# Autodesk Inventor assembly: RspCameraMia_cam_alone
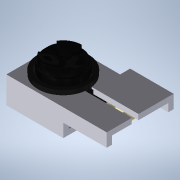
[picture p0: Inventor's stored thumbnail of the model, 180x180]
Saved by Autodesk Inventor 2020.2 (Build 242310000, 310)
## iProperties
Created: 2018-02-03
Part Number: RspCameraMia_cam_alone
Material: Genérico
Document SubType Name: Assembly
Designer: RafaX
Author: RafaX
## Documents named in this file (6)
- D:\gdrive\documents\flexipod\modelingv3\raspberry-pi-camera-module-v2-1\RspCameraMia_cam_alone.iam
- D:\gdrive\documents\flexipod\modelingv3\raspberry-pi-camera-module-v2-1\OVA5647_Housing.ipt
- D:\gdrive\documents\flexipod\modelingv3\raspberry-pi-camera-module-v2-1\OVA5647_Lens_FOV.ipt
- D:\gdrive\documents\flexipod\modelingv3\raspberry-pi-camera-module-v2-1\ribbon_cam.ipt
- D:\gdrive\documents\flexipod\modelingv3\raspberry-pi-camera-module-v2-1\CCD.ipt
- D:\gdrive\documents\flexipod\modelingv3\camera_cover.ipt
## Components (5 placed, 5 different names)
1. OVA5647_Housing:1 — Mate:1, Angle:1
2. OVA5647_Lens_FOV:1
3. ribbon_cam:1
4. CCD:1 — Flush:1
5. camera_cover:1 — Flush:1, Mate:1, Angle:1
## Relationships (3: Flush 1, Mate 1, Angle 1)
- Flush:1: CCD:1 ↔ camera_cover:1
- Mate:1: OVA5647_Housing:1 ↔ camera_cover:1
- Angle:1 (180 deg): OVA5647_Housing:1 ↔ camera_cover:1
